# Autodesk Inventor assembly: 4thRhinoRobot
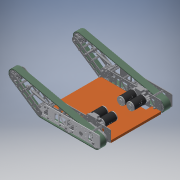
[picture p0: Inventor's stored thumbnail of the model, 180x180]
Saved by Autodesk Inventor 2016 SP1 (Build 200210100, 210)
## iProperties
Created: 2015-12-30
Part Number: 4thRhinoRobot
Document SubType Name: Assembly
Designer: steele
Mass: 23511.9 g
Surface Area: 38256.8 cm^2
Volume: 14882.3 cm^3
Density: 1.57986 g/cm^3
Author: steele
## Documents named in this file (5)
- C:\snobotics\CAD-Development\robSteele\SnoBotics2016\4thCutRhinoRobot\4thRhinoRobot.iam
- C:\snobotics\CAD-Development\robSteele\SnoBotics2016\RhinoTrackDrive\am-3322+RhinoTrackDriveModule.iam
- C:\snobotics\CAD-Development\robSteele\SnoBotics2016\FirstCutRhinoRobot\BasePlate.ipt
- C:\snobotics\CAD-Development\robSteele\SnoBotics2016\RhinoTrackDrive\am-3322+RhinoTrackDriveModule_MIR.iam
- C:\snobotics\autodesk\2015\FRC_KOP_2015\Motors\MOT_CIM-Motor_217-2000.iam
## Components (7 placed, 4 different names)
1. am-3322+RhinoTrackDriveModule:1 [sub-assembly] — Flush:1, Mate:2, Flush:2, Flush:3, Insert:1, Insert:2
2. BasePlate:1 — Mate:2, Flush:2, Flush:3, Flush:4, Flush:5
3. am-3322+RhinoTrackDriveModule_MIR:1 [sub-assembly] — Mate:1, Flush:4, Flush:5, Insert:3, Insert:4
4. MOT_CIM-Motor_217-2000:1 [sub-assembly] — Insert:1
5. MOT_CIM-Motor_217-2000:2 [sub-assembly] — Insert:2
6. MOT_CIM-Motor_217-2000:3 [sub-assembly] — Insert:3
7. MOT_CIM-Motor_217-2000:4 [sub-assembly] — Insert:4
## Relationships (11: Flush 5, Insert 4, Mate 2)
- Flush:1 (254 mm): am-3322+RhinoTrackDriveModule:1
- Mate:1 (165.1 mm): am-3322+RhinoTrackDriveModule_MIR:1
- Mate:2: am-3322+RhinoTrackDriveModule:1 ↔ BasePlate:1
- Flush:2: am-3322+RhinoTrackDriveModule:1 ↔ BasePlate:1
- Flush:3: am-3322+RhinoTrackDriveModule:1 ↔ BasePlate:1
- Flush:4: BasePlate:1 ↔ am-3322+RhinoTrackDriveModule_MIR:1
- Flush:5: BasePlate:1 ↔ am-3322+RhinoTrackDriveModule_MIR:1
- Insert:1: am-3322+RhinoTrackDriveModule:1 ↔ MOT_CIM-Motor_217-2000:1
- Insert:2: am-3322+RhinoTrackDriveModule:1 ↔ MOT_CIM-Motor_217-2000:2
- Insert:3: am-3322+RhinoTrackDriveModule_MIR:1 ↔ MOT_CIM-Motor_217-2000:3
- Insert:4: am-3322+RhinoTrackDriveModule_MIR:1 ↔ MOT_CIM-Motor_217-2000:4
## Named parameters: batteryWidth = 179.578 mm, centerOfBattery = 89.789 mm, widthOfRoboRIO = 146.1516 mm, centerOfRobotRIO = 73.0758 mm
